# Autodesk Inventor assembly: ModuleAssemblyV4
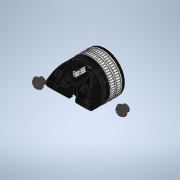
[picture p0: Inventor's stored thumbnail of the model, 180x180]
Saved by Autodesk Inventor 2020 (Build 240168000, 168)
## iProperties
Created: 2020-01-04
Part Number: ModuleAssemblyV4
Document SubType Name: Assembly
Designer: Connor
Author: Connor
## Documents named in this file (9)
- C:\Users\Connor\Documents\DifferentialSwerveV4\ModuleAssembly_V4.iam
- C:\Users\Connor\Documents\DifferentialSwerveV4\PlanetCarriage_V4.ipt
- C:\Users\Connor\Documents\DifferentialSwerveV4\RingGear_V4.iam
- C:\Users\Connor\Documents\DifferentialSwerveV4\BearingBall.ipt
- C:\Users\Connor\Documents\DifferentialSwerveV4\CarriageCap_V4.ipt
- C:\Users\Connor\Documents\GrabCAD\2019 Robot\Imported Components\Bearings\Radial_0.25x0.5x0.188.ipt
- C:\Users\Connor\Documents\DifferentialSwerveV4\Bevel15t.ipt
- C:\Users\Connor\Documents\DifferentialSwerveV4\WheelBracketHead_V4.ipt
- C:\Users\Connor\Documents\DifferentialSwerveV4\WheelBracketNut_V4.ipt
## Components (190 placed, 8 different names)
1. PlanetCarriage_V4:1 — Mate:1, Mate:2, Mate:3, Mate:5, Mate:6, Angle:1, Mate:7, Insert:3, Mate:8, Insert:4
2. RingGear_V4:1 [sub-assembly] — Mate:1, Mate:2, Mate:4, Tangent:2, Tangent:3
3. RingGear_V4:2 [sub-assembly] — Mate:3, Mate:4
4. CarriageCap_V4:1 — Mate:5, Mate:6, Angle:1, Insert:1, Insert:2
5. Radial_0.25x0.5x0.188:1 — Insert:1
6. Radial_0.25x0.5x0.188:2 — Insert:2
7. Bevel15t:1
8. Bevel15t:2
9. WheelBracketHead_V4:1 — Mate:7, Insert:3
10. WheelBracketNut_V4:1 — Mate:8, Insert:4
11. BearingBall:1 — Tangent:2, Tangent:3
12. BearingBall:2
13. BearingBall:3
14. BearingBall:4
15. BearingBall:5
16. BearingBall:6
17. BearingBall:7
18. BearingBall:8
19. BearingBall:9
20. BearingBall:10
21. BearingBall:11
22. BearingBall:12
23. BearingBall:13
24. BearingBall:14
25. BearingBall:15
26. BearingBall:16
27. BearingBall:17
28. BearingBall:18
29. BearingBall:19
30. BearingBall:20
31. BearingBall:21
32. BearingBall:22
33. BearingBall:23
34. BearingBall:24
35. BearingBall:25
36. BearingBall:26
37. BearingBall:27
38. BearingBall:28
39. BearingBall:29
40. BearingBall:30
41. BearingBall:31
42. BearingBall:32
43. BearingBall:33
44. BearingBall:34
45. BearingBall:35
46. BearingBall:36
47. BearingBall:37
48. BearingBall:38
49. BearingBall:39
50. BearingBall:40
51. BearingBall:41
52. BearingBall:42
53. BearingBall:43
54. BearingBall:44
55. BearingBall:45
56. BearingBall:46
57. BearingBall:47
58. BearingBall:48
59. BearingBall:49
60. BearingBall:50
61. BearingBall:51
62. BearingBall:52
63. BearingBall:53
64. BearingBall:54
65. BearingBall:55
66. BearingBall:56
67. BearingBall:57
68. BearingBall:58
69. BearingBall:59
70. BearingBall:60
71. BearingBall:61
72. BearingBall:62
73. BearingBall:63
74. BearingBall:64
75. BearingBall:65
76. BearingBall:66
77. BearingBall:67
78. BearingBall:68
79. BearingBall:69
80. BearingBall:70
81. BearingBall:71
82. BearingBall:72
83. BearingBall:73
84. BearingBall:74
85. BearingBall:75
86. BearingBall:76
87. BearingBall:77
88. BearingBall:78
89. BearingBall:79
90. BearingBall:80
91. BearingBall:81
92. BearingBall:82
93. BearingBall:83
94. BearingBall:84
95. BearingBall:85
96. BearingBall:86
97. BearingBall:87
98. BearingBall:88
99. BearingBall:89
100. BearingBall:90
101. BearingBall:91
102. BearingBall:92
103. BearingBall:93
104. BearingBall:94
105. BearingBall:95
106. BearingBall:96
107. BearingBall:97
108. BearingBall:98
109. BearingBall:99
110. BearingBall:100
111. BearingBall:101
112. BearingBall:102
113. BearingBall:103
114. BearingBall:104
115. BearingBall:105
116. BearingBall:106
117. BearingBall:107
118. BearingBall:108
119. BearingBall:109
120. BearingBall:110
121. BearingBall:111
122. BearingBall:112
123. BearingBall:113
124. BearingBall:114
125. BearingBall:115
126. BearingBall:116
127. BearingBall:117
128. BearingBall:118
129. BearingBall:119
130. BearingBall:120
131. BearingBall:121
132. BearingBall:122
133. BearingBall:123
134. BearingBall:124
135. BearingBall:125
136. BearingBall:126
137. BearingBall:127
138. BearingBall:128
139. BearingBall:129
140. BearingBall:130
141. BearingBall:131
142. BearingBall:132
143. BearingBall:133
144. BearingBall:134
145. BearingBall:135
146. BearingBall:136
147. BearingBall:137
148. BearingBall:138
149. BearingBall:139
150. BearingBall:140
151. BearingBall:141
152. BearingBall:142
153. BearingBall:143
154. BearingBall:144
155. BearingBall:145
156. BearingBall:146
157. BearingBall:147
158. BearingBall:148
159. BearingBall:149
160. BearingBall:150
161. BearingBall:151
162. BearingBall:152
163. BearingBall:153
164. BearingBall:154
165. BearingBall:155
166. BearingBall:156
167. BearingBall:157
168. BearingBall:158
169. BearingBall:159
170. BearingBall:160
171. BearingBall:161
172. BearingBall:162
173. BearingBall:163
174. BearingBall:164
175. BearingBall:165
176. BearingBall:166
177. BearingBall:167
178. BearingBall:168
179. BearingBall:169
180. BearingBall:170
181. BearingBall:171
182. BearingBall:172
183. BearingBall:173
184. BearingBall:174
185. BearingBall:175
186. BearingBall:176
187. BearingBall:177
188. BearingBall:178
189. BearingBall:179
190. BearingBall:180
## Component patterns: (3 elements), (60 elements, first: BearingBall:1), Component Pattern 3:2 (60 elements), Component Pattern 3:3 (60 elements)
## Relationships (15: Mate 8, Insert 4, Tangent 2, Angle 1)
- Mate:1: PlanetCarriage_V4:1 ↔ RingGear_V4:1
- Mate:2 (1.5875 mm): PlanetCarriage_V4:1 ↔ RingGear_V4:1
- Mate:3: PlanetCarriage_V4:1 ↔ RingGear_V4:2
- Mate:4 (1.5875 mm): RingGear_V4:1 ↔ RingGear_V4:2
- Tangent:2: RingGear_V4:1 ↔ BearingBall:1
- Tangent:3: RingGear_V4:1 ↔ BearingBall:1
- Mate:5: PlanetCarriage_V4:1 ↔ CarriageCap_V4:1
- Mate:6 (0.7937 mm): PlanetCarriage_V4:1 ↔ CarriageCap_V4:1
- Angle:1 (0 deg): PlanetCarriage_V4:1 ↔ CarriageCap_V4:1
- Insert:1: CarriageCap_V4:1 ↔ Radial_0.25x0.5x0.188:1
- Insert:2: CarriageCap_V4:1 ↔ Radial_0.25x0.5x0.188:2
- Mate:7: PlanetCarriage_V4:1 ↔ WheelBracketHead_V4:1
- Insert:3: PlanetCarriage_V4:1 ↔ WheelBracketHead_V4:1
- Mate:8: PlanetCarriage_V4:1 ↔ WheelBracketNut_V4:1
- Insert:4: PlanetCarriage_V4:1 ↔ WheelBracketNut_V4:1
